# Autodesk Inventor assembly: Flex
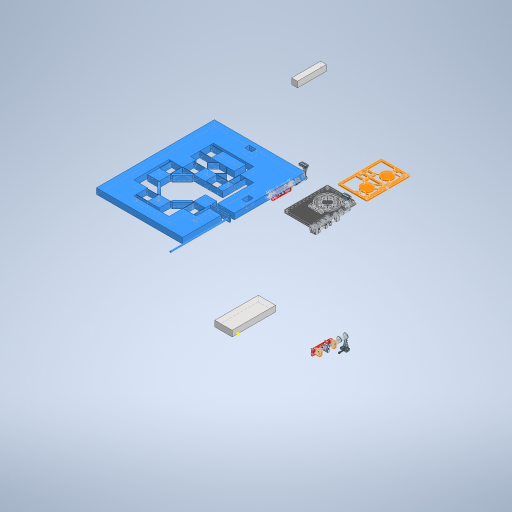
[picture p0: Inventor's stored thumbnail of the model, 512x512]
Saved by Autodesk Inventor 2023 (Build 270158000, 158)
## iProperties
Created: 2023-03-17
Part Number: Flex
Document SubType Name: Assembly
Designer: Nathann
Author: Nathann
## Documents named in this file (34)
- C:\Users\Nathann\OneDrive\ClawdDrive\Objet3D\IminaProbe\Flex.iam
- C:\Users\Nathann\OneDrive\ClawdDrive\Objet3D\IminaProbe\FlexBlocK7.ipt
- C:\Users\Nathann\OneDrive\ClawdDrive\Objet3D\IminaProbe\FlexBlocWheel.ipt
- C:\Users\Nathann\OneDrive\ClawdDrive\Objet3D\IminaProbe\Part1.ipt
- C:\Users\Nathann\OneDrive\ClawdDrive\Objet3D\IminaProbe\FlexBlockWheelSupport.ipt
- C:\Users\Nathann\OneDrive\ClawdDrive\Objet3D\IminaProbe\FlexBlocTristan.ipt
- C:\Users\Nathann\OneDrive\ClawdDrive\Objet3D\IminaProbe\motorAxis.ipt
- C:\Users\Nathann\OneDrive\ClawdDrive\Objet3D\LEMARUAG\GP16A_2-Stufig-110322.ipt
- C:\Users\Nathann\OneDrive\ClawdDrive\Objet3D\LEMARUAG\283825_ec-max16_5w.ipt
- C:\Users\Nathann\OneDrive\ClawdDrive\Objet3D\IminaProbe\4145N198_Set Screw Precision Flexible Shaft Couplings.ipt
- C:\Users\Nathann\OneDrive\ClawdDrive\Objet3D\IminaProbe\90751A114_18-8 Stainless Steel Socket Head Screws.ipt
- C:\Users\Nathann\OneDrive\ClawdDrive\Objet3D\IminaProbe\94450A564_Left-Hand Threaded 18-8 Stainless Steel Thin Hex Nut.ipt
- C:\Users\Nathann\OneDrive\ClawdDrive\Objet3D\IminaProbe\91292A832_18-8 Stainless Steel Socket Head Screw.ipt
- C:\Users\Nathann\OneDrive\ClawdDrive\Objet3D\IminaProbe\POMSliderMotor.ipt
- C:\Users\Nathann\OneDrive\ClawdDrive\Objet3D\IminaProbe\MotorMountDifferential.ipt
- C:\Users\Nathann\OneDrive\ClawdDrive\Objet3D\IminaProbe\93805A627_18-8 Stainless Steel Threaded Rod.ipt
- C:\Users\Nathann\OneDrive\ClawdDrive\Objet3D\IminaProbe\93805A631_18-8 Stainless Steel Threaded Rod.ipt
- C:\Users\Nathann\OneDrive\ClawdDrive\Objet3D\IminaProbe\91828A113_18-8 Stainless Steel Hex Nut.ipt
- C:\Users\Nathann\OneDrive\ClawdDrive\Objet3D\IminaProbe\MotorDifferentialMountingBracket.ipt
- C:\Users\Nathann\OneDrive\ClawdDrive\Objet3D\IminaProbe\POMSliderMotorM25.ipt
- C:\Users\Nathann\OneDrive\ClawdDrive\Objet3D\IminaProbe\SliderFixtureM25.ipt
- C:\Users\Nathann\OneDrive\ClawdDrive\Objet3D\IminaProbe\AxisJoinerThreaded.ipt
- C:\Users\Nathann\OneDrive\ClawdDrive\Objet3D\IminaProbe\AxisLinear.ipt
- C:\Users\Nathann\OneDrive\ClawdDrive\Objet3D\IminaProbe\POMSliderAxis.ipt
- C:\Users\Nathann\OneDrive\ClawdDrive\Objet3D\IminaProbe\TigeM3FinAxis.ipt
- C:\Users\Nathann\OneDrive\ClawdDrive\Objet3D\IminaProbe\AxisLinearShort.ipt
- C:\Users\Nathann\OneDrive\ClawdDrive\Objet3D\IminaProbe\MotorlMountingBracket.ipt
- C:\Users\Nathann\OneDrive\ClawdDrive\Objet3D\IminaProbe\FlexK7V2.ipt
- C:\Users\Nathann\OneDrive\ClawdDrive\Objet3D\IminaProbe\Flex\AIP\FEA\ea0gbbme8.fins
- C:\Users\Nathann\OneDrive\ClawdDrive\Objet3D\IminaProbe\Flex\AIP\FEA\ea0gbbme8.fsat
- C:\Users\Nathann\OneDrive\ClawdDrive\Objet3D\IminaProbe\Flex\AIP\FEA\ea0gbbme8.ftes
- C:\Users\Nathann\OneDrive\ClawdDrive\Objet3D\IminaProbe\Flex\AIP\FEA\ea0gbbme8.fwiz
- C:\Users\Nathann\OneDrive\ClawdDrive\Objet3D\IminaProbe\Flex\AIP\FEA\ea0gbbmf4.fmsh
- C:\Users\Nathann\OneDrive\ClawdDrive\Objet3D\IminaProbe\Flex\AIP\FEA\ea0gbbmf5.fres
## Components (113 placed, 27 different names)
1. FlexBlocK7:1
2. FlexBlocWheel:1 — Flush:1, Flush:2, Mate:1
3. Part1:1
4. FlexBlockWheelSupport:1 — Flush:1, Flush:2, Mate:1
5. FlexBlocTristan:1
6. motorAxis:1
7. GP16A_2-Stufig-110322:2 — Insert:23, Insert:24
8. 283825_ec-max16_5w:2
9. 4145N198_Set Screw Precision Flexible Shaft Couplings:2 — Insert:27
10. 91292A832_18-8 Stainless Steel Socket Head Screw:5 — Insert:28
11. 91292A832_18-8 Stainless Steel Socket Head Screw:6 — Insert:29
12. MotorMountDifferential:1 — Insert:23, Insert:24, Insert:28, Insert:29, Flush:10, Flush:12, Flush:13, Insert:43, Insert:44, Insert:45, Insert:46
13. 93805A627_18-8 Stainless Steel Threaded Rod:1 — Insert:26, Rotation:1
14. 93805A631_18-8 Stainless Steel Threaded Rod:2 — Insert:26, Insert:27, Insert:41, Rotation:1
15. 91828A113_18-8 Stainless Steel Hex Nut:1 — Mate:26, Mate:27, Mate:28
16. 94450A564_Left-Hand Threaded 18-8 Stainless Steel Thin Hex Nut:3 — Mate:21, Mate:22, Mate:23
17. MotorDifferentialMountingBracket:1 — Insert:30, Insert:31, Insert:32, Insert:33, Flush:14, Flush:15, Mate:25, Insert:34, Insert:35, Insert:36, Insert:37, Flush:16, Mate:29, Flush:17
18. POMSliderMotorM25:1 — Mate:15, Flush:9, Flush:10, Flush:11, Mate:26, Mate:27, Mate:28, Insert:52, Flush:26
19. SliderFixtureM25:1 — Mate:15, Flush:9, Flush:11, Insert:38, Insert:39, Flush:17
20. POMSliderMotor:3 — Flush:12, Flush:14, Flush:15, Mate:25, Insert:53
21. POMSliderMotor:4 — Flush:13, Mate:21, Mate:22, Mate:23, Flush:16, Mate:29, Insert:51
22. 91292A832_18-8 Stainless Steel Socket Head Screw:9 — Insert:31
23. 91292A832_18-8 Stainless Steel Socket Head Screw:10 — Insert:30
24. 91292A832_18-8 Stainless Steel Socket Head Screw:11 — Insert:33
25. 91292A832_18-8 Stainless Steel Socket Head Screw:12 — Insert:32
26. 91292A832_18-8 Stainless Steel Socket Head Screw:13 — Insert:36
27. 91292A832_18-8 Stainless Steel Socket Head Screw:14 — Insert:34
28. 91292A832_18-8 Stainless Steel Socket Head Screw:15 — Insert:37
29. 91292A832_18-8 Stainless Steel Socket Head Screw:16 — Insert:35
30. 91292A832_18-8 Stainless Steel Socket Head Screw:17 — Insert:39
31. 91292A832_18-8 Stainless Steel Socket Head Screw:18 — Insert:38
32. AxisJoinerThreaded:2 — Insert:41
33. AxisLinear:1 — Insert:43, Insert:47
34. AxisLinear:2 — Insert:44, Insert:48
35. 91292A832_18-8 Stainless Steel Socket Head Screw:19 — Insert:46
36. 91292A832_18-8 Stainless Steel Socket Head Screw:20 — Insert:45
37. MotorMountDifferential:2 — Insert:47, Insert:48, Insert:49, Insert:50, Flush:18
38. 91292A832_18-8 Stainless Steel Socket Head Screw:21 — Insert:49
39. 91292A832_18-8 Stainless Steel Socket Head Screw:22 — Insert:50
40. POMSliderAxis:1 — Insert:52, Insert:55, Flush:26
41. POMSliderAxis:2 — Insert:53, Insert:56, Flush:18
42. POMSliderAxis:3 — Insert:51, Insert:54
43. 91292A832_18-8 Stainless Steel Socket Head Screw:23 — Insert:56
44. 91292A832_18-8 Stainless Steel Socket Head Screw:24 — Insert:55
45. 91292A832_18-8 Stainless Steel Socket Head Screw:25 — Insert:54
46. GP16A_2-Stufig-110322:3
47. 283825_ec-max16_5w:3
48. 4145N198_Set Screw Precision Flexible Shaft Couplings:3 — Insert:89
49. 91292A832_18-8 Stainless Steel Socket Head Screw:26
50. 91292A832_18-8 Stainless Steel Socket Head Screw:27
51. MotorMountDifferential:3 — Insert:90
52. 91828A113_18-8 Stainless Steel Hex Nut:2
53. POMSliderMotorM25:2 — Mate:38, Flush:22
54. SliderFixtureM25:2 — Flush:24
55. 91292A832_18-8 Stainless Steel Socket Head Screw:36
56. 91292A832_18-8 Stainless Steel Socket Head Screw:37
57. 91292A832_18-8 Stainless Steel Socket Head Screw:39
58. MotorMountDifferential:4 — Insert:92, Flush:23, Flush:25
59. 91292A832_18-8 Stainless Steel Socket Head Screw:41
60. POMSliderAxis:5 — Flush:22
61. 91292A832_18-8 Stainless Steel Socket Head Screw:43
62. TigeM3FinAxis:1 — Insert:89
63. AxisLinearShort:1 — Insert:90, Insert:92, Mate:38
64. 90751A114_18-8 Stainless Steel Socket Head Screws:1
65. MotorlMountingBracket:1 — Flush:23, Flush:24, Flush:25, Insert:93, Insert:94, Insert:95, Insert:96, Insert:97, Insert:98, Insert:99, Insert:100
66. 91292A832_18-8 Stainless Steel Socket Head Screw:44 — Insert:93, Mate:39
67. 91292A832_18-8 Stainless Steel Socket Head Screw:45 — Insert:96
68. 91292A832_18-8 Stainless Steel Socket Head Screw:46 — Insert:94
69. 91292A832_18-8 Stainless Steel Socket Head Screw:47 — Insert:95
70. 91292A832_18-8 Stainless Steel Socket Head Screw:48 — Insert:97
71. 91292A832_18-8 Stainless Steel Socket Head Screw:49 — Insert:98
72. 91292A832_18-8 Stainless Steel Socket Head Screw:50 — Insert:100
73. 91292A832_18-8 Stainless Steel Socket Head Screw:51 — Insert:99
74. GP16A_2-Stufig-110322:4
75. 283825_ec-max16_5w:4
76. 4145N198_Set Screw Precision Flexible Shaft Couplings:4
77. 91292A832_18-8 Stainless Steel Socket Head Screw:52
78. 91292A832_18-8 Stainless Steel Socket Head Screw:53
79. MotorMountDifferential:5
80. 93805A627_18-8 Stainless Steel Threaded Rod:2
81. 93805A631_18-8 Stainless Steel Threaded Rod:3
82. 91828A113_18-8 Stainless Steel Hex Nut:3
83. 94450A564_Left-Hand Threaded 18-8 Stainless Steel Thin Hex Nut:4
84. MotorDifferentialMountingBracket:2
85. POMSliderMotorM25:3
86. SliderFixtureM25:3
87. POMSliderMotor:5
88. POMSliderMotor:6
89. 91292A832_18-8 Stainless Steel Socket Head Screw:54
90. 91292A832_18-8 Stainless Steel Socket Head Screw:55
91. 91292A832_18-8 Stainless Steel Socket Head Screw:56
92. 91292A832_18-8 Stainless Steel Socket Head Screw:57
93. 91292A832_18-8 Stainless Steel Socket Head Screw:58
94. 91292A832_18-8 Stainless Steel Socket Head Screw:59
95. 91292A832_18-8 Stainless Steel Socket Head Screw:60
96. 91292A832_18-8 Stainless Steel Socket Head Screw:61
97. 91292A832_18-8 Stainless Steel Socket Head Screw:62
98. 91292A832_18-8 Stainless Steel Socket Head Screw:63
99. AxisJoinerThreaded:3
100. AxisLinear:3
101. AxisLinear:4
102. 91292A832_18-8 Stainless Steel Socket Head Screw:64
103. 91292A832_18-8 Stainless Steel Socket Head Screw:65
104. MotorMountDifferential:6
105. 91292A832_18-8 Stainless Steel Socket Head Screw:66
106. 91292A832_18-8 Stainless Steel Socket Head Screw:67
107. POMSliderAxis:6
108. POMSliderAxis:7
109. POMSliderAxis:8
110. 91292A832_18-8 Stainless Steel Socket Head Screw:68
111. 91292A832_18-8 Stainless Steel Socket Head Screw:69
112. 91292A832_18-8 Stainless Steel Socket Head Screw:70
113. FlexK7V2:1
## Relationships (147: Insert 89, Flush 31, Mate 25, RelateRotation 2)
- Flush:1: FlexBlocWheel:1 ↔ FlexBlockWheelSupport:1
- Flush:2: FlexBlocWheel:1 ↔ FlexBlockWheelSupport:1
- Mate:1: FlexBlocWheel:1 ↔ FlexBlockWheelSupport:1
- [Insert]: GP16A_2-Stufig-110322:2 ↔ 283825_ec-max16_5w:2
- [Insert] (-4 mm): GP16A_2-Stufig-110322:2 ↔ 4145N198_Set Screw Precision Flexible Shaft Couplings:2
- Insert:23: GP16A_2-Stufig-110322:2 ↔ MotorMountDifferential:1
- Insert:24: GP16A_2-Stufig-110322:2 ↔ MotorMountDifferential:1
- Insert:26: 93805A627_18-8 Stainless Steel Threaded Rod:1 ↔ 93805A631_18-8 Stainless Steel Threaded Rod:2
- Insert:27 (-4 mm): 4145N198_Set Screw Precision Flexible Shaft Couplings:2 ↔ 93805A631_18-8 Stainless Steel Threaded Rod:2
- Insert:28: 91292A832_18-8 Stainless Steel Socket Head Screw:5 ↔ MotorMountDifferential:1
- Insert:29: 91292A832_18-8 Stainless Steel Socket Head Screw:6 ↔ MotorMountDifferential:1
- Mate:15: POMSliderMotorM25:1 ↔ SliderFixtureM25:1
- Flush:9: POMSliderMotorM25:1 ↔ SliderFixtureM25:1
- Flush:10: MotorMountDifferential:1 ↔ POMSliderMotorM25:1
- Flush:11: POMSliderMotorM25:1 ↔ SliderFixtureM25:1
- Flush:12: MotorMountDifferential:1 ↔ POMSliderMotor:3
- Flush:13: MotorMountDifferential:1 ↔ POMSliderMotor:4
- Mate:21: 94450A564_Left-Hand Threaded 18-8 Stainless Steel Thin Hex Nut:3 ↔ POMSliderMotor:4
- Mate:22: 94450A564_Left-Hand Threaded 18-8 Stainless Steel Thin Hex Nut:3 ↔ POMSliderMotor:4
- Mate:23: 94450A564_Left-Hand Threaded 18-8 Stainless Steel Thin Hex Nut:3 ↔ POMSliderMotor:4
- Insert:30: MotorDifferentialMountingBracket:1 ↔ 91292A832_18-8 Stainless Steel Socket Head Screw:10
- Insert:31: MotorDifferentialMountingBracket:1 ↔ 91292A832_18-8 Stainless Steel Socket Head Screw:9
- Insert:32: MotorDifferentialMountingBracket:1 ↔ 91292A832_18-8 Stainless Steel Socket Head Screw:12
- Insert:33: MotorDifferentialMountingBracket:1 ↔ 91292A832_18-8 Stainless Steel Socket Head Screw:11
- Flush:14: MotorDifferentialMountingBracket:1 ↔ POMSliderMotor:3
- Flush:15: MotorDifferentialMountingBracket:1 ↔ POMSliderMotor:3
- Mate:25: MotorDifferentialMountingBracket:1 ↔ POMSliderMotor:3
- Insert:34: MotorDifferentialMountingBracket:1 ↔ 91292A832_18-8 Stainless Steel Socket Head Screw:14
- Insert:35: MotorDifferentialMountingBracket:1 ↔ 91292A832_18-8 Stainless Steel Socket Head Screw:16
- Insert:36: MotorDifferentialMountingBracket:1 ↔ 91292A832_18-8 Stainless Steel Socket Head Screw:13
- Insert:37: MotorDifferentialMountingBracket:1 ↔ 91292A832_18-8 Stainless Steel Socket Head Screw:15
- Flush:16: MotorDifferentialMountingBracket:1 ↔ POMSliderMotor:4
- Insert:38: SliderFixtureM25:1 ↔ 91292A832_18-8 Stainless Steel Socket Head Screw:18
- Insert:39: SliderFixtureM25:1 ↔ 91292A832_18-8 Stainless Steel Socket Head Screw:17
- Insert:41 (-3 mm): 93805A631_18-8 Stainless Steel Threaded Rod:2 ↔ AxisJoinerThreaded:2
- Mate:26: 91828A113_18-8 Stainless Steel Hex Nut:1 ↔ POMSliderMotorM25:1
- Mate:27: 91828A113_18-8 Stainless Steel Hex Nut:1 ↔ POMSliderMotorM25:1
- Mate:28: 91828A113_18-8 Stainless Steel Hex Nut:1 ↔ POMSliderMotorM25:1
- Rotation:1 [RelateRotation] (1 ul): 93805A627_18-8 Stainless Steel Threaded Rod:1 ↔ 93805A631_18-8 Stainless Steel Threaded Rod:2
- Insert:43: MotorMountDifferential:1 ↔ AxisLinear:1
- Insert:44: MotorMountDifferential:1 ↔ AxisLinear:2
- Insert:45: MotorMountDifferential:1 ↔ 91292A832_18-8 Stainless Steel Socket Head Screw:20
- Insert:46: MotorMountDifferential:1 ↔ 91292A832_18-8 Stainless Steel Socket Head Screw:19
- Insert:47: AxisLinear:1 ↔ MotorMountDifferential:2
- Insert:48: AxisLinear:2 ↔ MotorMountDifferential:2
- Insert:49: MotorMountDifferential:2 ↔ 91292A832_18-8 Stainless Steel Socket Head Screw:21
- Insert:50: MotorMountDifferential:2 ↔ 91292A832_18-8 Stainless Steel Socket Head Screw:22
- Mate:29: MotorDifferentialMountingBracket:1 ↔ POMSliderMotor:4
- Insert:51: POMSliderMotor:4 ↔ POMSliderAxis:3
- Insert:52: POMSliderMotorM25:1 ↔ POMSliderAxis:1
- Insert:53: POMSliderMotor:3 ↔ POMSliderAxis:2
- Insert:54: POMSliderAxis:3 ↔ 91292A832_18-8 Stainless Steel Socket Head Screw:25
- Insert:55: POMSliderAxis:1 ↔ 91292A832_18-8 Stainless Steel Socket Head Screw:24
- Insert:56: POMSliderAxis:2 ↔ 91292A832_18-8 Stainless Steel Socket Head Screw:23
- Flush:17: MotorDifferentialMountingBracket:1 ↔ SliderFixtureM25:1
- Flush:18: MotorMountDifferential:2 ↔ POMSliderAxis:2
- [Insert]: GP16A_2-Stufig-110322:3 ↔ 283825_ec-max16_5w:3
- [Insert] (-4 mm): GP16A_2-Stufig-110322:3 ↔ 4145N198_Set Screw Precision Flexible Shaft Couplings:3
- [Insert]: GP16A_2-Stufig-110322:3 ↔ MotorMountDifferential:3
- [Insert]: GP16A_2-Stufig-110322:3 ↔ MotorMountDifferential:3
- [Insert]: 91292A832_18-8 Stainless Steel Socket Head Screw:26 ↔ MotorMountDifferential:3
- [Insert]: 91292A832_18-8 Stainless Steel Socket Head Screw:27 ↔ MotorMountDifferential:3
- [Mate]: POMSliderMotorM25:2 ↔ SliderFixtureM25:2
- [Flush]: POMSliderMotorM25:2 ↔ SliderFixtureM25:2
- [Flush]: MotorMountDifferential:3 ↔ POMSliderMotorM25:2
- [Flush]: POMSliderMotorM25:2 ↔ SliderFixtureM25:2
- [Insert]: SliderFixtureM25:2 ↔ 91292A832_18-8 Stainless Steel Socket Head Screw:37
- [Insert]: SliderFixtureM25:2 ↔ 91292A832_18-8 Stainless Steel Socket Head Screw:36
- [Mate]: 91828A113_18-8 Stainless Steel Hex Nut:2 ↔ POMSliderMotorM25:2
- [Mate]: 91828A113_18-8 Stainless Steel Hex Nut:2 ↔ POMSliderMotorM25:2
- [Mate]: 91828A113_18-8 Stainless Steel Hex Nut:2 ↔ POMSliderMotorM25:2
- [Insert]: MotorMountDifferential:3 ↔ 91292A832_18-8 Stainless Steel Socket Head Screw:39
- [Insert]: MotorMountDifferential:4 ↔ 91292A832_18-8 Stainless Steel Socket Head Screw:41
- [Insert]: POMSliderMotorM25:2 ↔ POMSliderAxis:5
- [Insert]: POMSliderAxis:5 ↔ 91292A832_18-8 Stainless Steel Socket Head Screw:43
- Insert:89 (-4 mm): 4145N198_Set Screw Precision Flexible Shaft Couplings:3 ↔ TigeM3FinAxis:1
- Insert:90: MotorMountDifferential:3 ↔ AxisLinearShort:1
- Insert:92: MotorMountDifferential:4 ↔ AxisLinearShort:1
- Mate:38: POMSliderMotorM25:2 ↔ AxisLinearShort:1
- Flush:22: POMSliderMotorM25:2 ↔ POMSliderAxis:5
- Flush:23: MotorMountDifferential:4 ↔ MotorlMountingBracket:1
- Flush:24: SliderFixtureM25:2 ↔ MotorlMountingBracket:1
- Flush:25: MotorMountDifferential:4 ↔ MotorlMountingBracket:1
- Insert:93: MotorlMountingBracket:1 ↔ 91292A832_18-8 Stainless Steel Socket Head Screw:44
- Mate:39: 91292A832_18-8 Stainless Steel Socket Head Screw:44
- Insert:94: MotorlMountingBracket:1 ↔ 91292A832_18-8 Stainless Steel Socket Head Screw:46
- Insert:95: MotorlMountingBracket:1 ↔ 91292A832_18-8 Stainless Steel Socket Head Screw:47
- Insert:96: MotorlMountingBracket:1 ↔ 91292A832_18-8 Stainless Steel Socket Head Screw:45
- Insert:97: MotorlMountingBracket:1 ↔ 91292A832_18-8 Stainless Steel Socket Head Screw:48
- Insert:98: MotorlMountingBracket:1 ↔ 91292A832_18-8 Stainless Steel Socket Head Screw:49
- Insert:99: MotorlMountingBracket:1 ↔ 91292A832_18-8 Stainless Steel Socket Head Screw:51
- Insert:100: MotorlMountingBracket:1 ↔ 91292A832_18-8 Stainless Steel Socket Head Screw:50
- Flush:26: POMSliderMotorM25:1 ↔ POMSliderAxis:1
- [Insert]: GP16A_2-Stufig-110322:4 ↔ 283825_ec-max16_5w:4
- [Insert] (-4 mm): GP16A_2-Stufig-110322:4 ↔ 4145N198_Set Screw Precision Flexible Shaft Couplings:4
- [Insert]: GP16A_2-Stufig-110322:4 ↔ MotorMountDifferential:5
- [Insert]: GP16A_2-Stufig-110322:4 ↔ MotorMountDifferential:5
- [Insert]: 93805A627_18-8 Stainless Steel Threaded Rod:2 ↔ 93805A631_18-8 Stainless Steel Threaded Rod:3
- [Insert] (-4 mm): 4145N198_Set Screw Precision Flexible Shaft Couplings:4 ↔ 93805A631_18-8 Stainless Steel Threaded Rod:3
- [Insert]: 91292A832_18-8 Stainless Steel Socket Head Screw:52 ↔ MotorMountDifferential:5
- [Insert]: 91292A832_18-8 Stainless Steel Socket Head Screw:53 ↔ MotorMountDifferential:5
- [Mate]: POMSliderMotorM25:3 ↔ SliderFixtureM25:3
- [Flush]: POMSliderMotorM25:3 ↔ SliderFixtureM25:3
- [Flush]: MotorMountDifferential:5 ↔ POMSliderMotorM25:3
- [Flush]: POMSliderMotorM25:3 ↔ SliderFixtureM25:3
- [Flush]: MotorMountDifferential:5 ↔ POMSliderMotor:5
- [Flush]: MotorMountDifferential:5 ↔ POMSliderMotor:6
- [Mate]: 94450A564_Left-Hand Threaded 18-8 Stainless Steel Thin Hex Nut:4 ↔ POMSliderMotor:6
- [Mate]: 94450A564_Left-Hand Threaded 18-8 Stainless Steel Thin Hex Nut:4 ↔ POMSliderMotor:6
- [Mate]: 94450A564_Left-Hand Threaded 18-8 Stainless Steel Thin Hex Nut:4 ↔ POMSliderMotor:6
- [Insert]: MotorDifferentialMountingBracket:2 ↔ 91292A832_18-8 Stainless Steel Socket Head Screw:55
- [Insert]: MotorDifferentialMountingBracket:2 ↔ 91292A832_18-8 Stainless Steel Socket Head Screw:54
- [Insert]: MotorDifferentialMountingBracket:2 ↔ 91292A832_18-8 Stainless Steel Socket Head Screw:57
- [Insert]: MotorDifferentialMountingBracket:2 ↔ 91292A832_18-8 Stainless Steel Socket Head Screw:56
- [Flush]: MotorDifferentialMountingBracket:2 ↔ POMSliderMotor:5
- [Flush]: MotorDifferentialMountingBracket:2 ↔ POMSliderMotor:5
- [Mate]: MotorDifferentialMountingBracket:2 ↔ POMSliderMotor:5
- [Insert]: MotorDifferentialMountingBracket:2 ↔ 91292A832_18-8 Stainless Steel Socket Head Screw:59
- [Insert]: MotorDifferentialMountingBracket:2 ↔ 91292A832_18-8 Stainless Steel Socket Head Screw:61
- [Insert]: MotorDifferentialMountingBracket:2 ↔ 91292A832_18-8 Stainless Steel Socket Head Screw:58
- [Insert]: MotorDifferentialMountingBracket:2 ↔ 91292A832_18-8 Stainless Steel Socket Head Screw:60
- [Flush]: MotorDifferentialMountingBracket:2 ↔ POMSliderMotor:6
- [Insert]: SliderFixtureM25:3 ↔ 91292A832_18-8 Stainless Steel Socket Head Screw:63
- [Insert]: SliderFixtureM25:3 ↔ 91292A832_18-8 Stainless Steel Socket Head Screw:62
- [Insert] (-3 mm): 93805A631_18-8 Stainless Steel Threaded Rod:3 ↔ AxisJoinerThreaded:3
- [Mate]: 91828A113_18-8 Stainless Steel Hex Nut:3 ↔ POMSliderMotorM25:3
- [Mate]: 91828A113_18-8 Stainless Steel Hex Nut:3 ↔ POMSliderMotorM25:3
- [Mate]: 91828A113_18-8 Stainless Steel Hex Nut:3 ↔ POMSliderMotorM25:3
- [RelateRotation] (1 ul): 93805A627_18-8 Stainless Steel Threaded Rod:2 ↔ 93805A631_18-8 Stainless Steel Threaded Rod:3
- [Insert]: MotorMountDifferential:5 ↔ AxisLinear:3
- [Insert]: MotorMountDifferential:5 ↔ AxisLinear:4
- [Insert]: MotorMountDifferential:5 ↔ 91292A832_18-8 Stainless Steel Socket Head Screw:65
- [Insert]: MotorMountDifferential:5 ↔ 91292A832_18-8 Stainless Steel Socket Head Screw:64
- [Insert]: AxisLinear:3 ↔ MotorMountDifferential:6
- [Insert]: AxisLinear:4 ↔ MotorMountDifferential:6
- [Insert]: MotorMountDifferential:6 ↔ 91292A832_18-8 Stainless Steel Socket Head Screw:66
- [Insert]: MotorMountDifferential:6 ↔ 91292A832_18-8 Stainless Steel Socket Head Screw:67
- [Mate]: MotorDifferentialMountingBracket:2 ↔ POMSliderMotor:6
- [Insert]: POMSliderMotor:6 ↔ POMSliderAxis:8
- [Insert]: POMSliderMotorM25:3 ↔ POMSliderAxis:6
- [Insert]: POMSliderMotor:5 ↔ POMSliderAxis:7
- [Insert]: POMSliderAxis:8 ↔ 91292A832_18-8 Stainless Steel Socket Head Screw:70
- [Insert]: POMSliderAxis:6 ↔ 91292A832_18-8 Stainless Steel Socket Head Screw:69
- [Insert]: POMSliderAxis:7 ↔ 91292A832_18-8 Stainless Steel Socket Head Screw:68
- [Flush]: MotorDifferentialMountingBracket:2 ↔ SliderFixtureM25:3
- [Flush]: MotorMountDifferential:6 ↔ POMSliderAxis:7
- [Flush]: POMSliderMotorM25:3 ↔ POMSliderAxis:6
## Named parameters: sa_0 = 1, d33_d3 = 0 mm, d43_d9 = -4 mm, d137_d131 = 0 mm, d141_d105 = 0 mm, d142_d106 = 0 mm, d143_d107 = 0 mm, d147_d120 = 0 mm, d152_d125 = 0 mm, d155_d128 = 0 mm, d157_d73 = 0 mm, d158_d75 = 0 mm, d159_d76 = 0 mm, d177_d101 = 0 mm, d178_d102 = 0 mm, d180_d33_d3 = 0 mm, d181_d43_d9 = -4 mm, d182_d54 = 0 mm, d183_d55 = 0 mm, d186_d67 = 0 mm, d187_d68 = 0 mm, d188_d72 = 0 mm, d215_d130 = 0 mm, d216_d131 = 0 mm, d217_d132 = 0 mm, d218_d133 = 0 mm, d219_d134 = 0 mm, d220_d105 = 0 mm, d221_d106 = 0 mm, d222_d107 = 0 mm, d223_d116 = 1, d224_d118 = 0 mm, d225_d119 = 0 mm, d226_d120 = 0 mm, d227_d121 = 0 mm, d228_d122 = 0 mm, d229_d123 = 0 mm, d230_d124 = 0 mm, d231_d125 = 0 mm, d232_d126 = 0 mm, d233_d127 = 0 mm, d234_d128 = 0 mm, d235_d129 = 0 mm, d236_d73 = 0 mm, d237_d75 = 0 mm, d238_d76 = 0 mm, d239_d77 = 0 mm, d240_d78 = 0 mm, d241_d83 = 0 mm, d242_d84 = 0 mm, d243_d85 = 0 mm, d244_d87 = 0 mm, d245_d88 = 0 mm, d246_d89 = 0 mm, d247_d90 = 0 mm, d248_d91 = 0 mm, d249_d92 = 0 mm, d250_d93 = 0 mm, d251_d94 = 0 mm, d252_d95 = 0 mm, d253_d96 = 0 mm, d254_d97 = 0 mm, d255_d98 = 0 mm, d256_d101 = 0 mm, d257_d102 = 0 mm, d258_d104 = -3 mm, d259_d33_d3 = 0 mm, d260_d43_d9 = -4 mm, d261_d54 = 0 mm, d262_d55 = 0 mm, d263_d65 = 0 mm, d264_d66 = -4 mm, d265_d67 = 0 mm, d266_d68 = 0 mm, d267_d72 = 0 mm, d268_d214 = 0 mm
note: some values were not read from the file. Shown as the stored number, unit unknown: "sa_0".
